# Autodesk Inventor assembly: mg996 3mm top
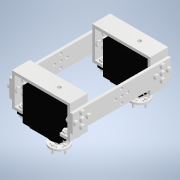
[picture p0: Inventor's stored thumbnail of the model, 180x180]
Saved by Autodesk Inventor 2021.4 (Build 254397000, 397)
## iProperties
Created: 2022-07-09
Part Number: mg996 3mm top
Document SubType Name: Assembly
Designer: isamu
Author: isamu
## Documents named in this file (5)
- D:\personal_projects\robot\inventor\2021\mg996 3mm top.iam
- D:\personal_projects\robot\inventor\2021\base mg996r 3mm frame.iam
- D:\personal_projects\robot\exports\frames\servo frame part 4.ipt
- D:\personal_projects\robot\exports\screws\m3x8.ipt
- D:\personal_projects\robot\exports\screws\m3 nuts.ipt
## Components (44 placed, 4 different names)
1. base mg996r 3mm frame:1 [sub-assembly] — Mate:4, Mate:5, Mate:6, Mate:7, Mate:8, Insert:26, Insert:27, Insert:28, Insert:29, Insert:30, Insert:36, Insert:37, Insert:38, Insert:39, Insert:40
2. base mg996r 3mm frame:2 [sub-assembly] — Mate:1, Mate:2, Mate:3, Mate:9, Mate:10, Mate:11, Insert:21, Insert:22, Insert:23, Insert:24, Insert:25, Insert:31, Insert:32, Insert:33, Insert:34, Insert:35
3. servo frame part 4:1 — Mate:1, Mate:2, Mate:3, Mate:4, Mate:5, Mate:6, Insert:1, Insert:2, Insert:3, Insert:4, Insert:5, Insert:6, Insert:7, Insert:8, Insert:9, Insert:10
4. servo frame part 4:2 — Mate:7, Mate:8, Mate:9, Mate:10, Mate:11, Insert:11, Insert:12, Insert:13, Insert:14, Insert:15, Insert:16, Insert:17, Insert:18, Insert:19, Insert:20
5. m3x8:1 — Insert:5
6. m3x8:2 — Insert:3
7. m3x8:3 — Insert:4
8. m3x8:4 — Insert:1
9. m3x8:5 — Insert:2
10. m3x8:6 — Insert:6
11. m3x8:7 — Insert:7
12. m3x8:8 — Insert:8
13. m3x8:9 — Insert:9
14. m3x8:10 — Insert:10
15. m3x8:11 — Insert:11
16. m3x8:12 — Insert:12
17. m3x8:13 — Insert:13
18. m3x8:14 — Insert:14
19. m3x8:15 — Insert:15
20. m3x8:16 — Insert:17
21. m3x8:17 — Insert:18
22. m3x8:18 — Insert:19
23. m3x8:19 — Insert:20
24. m3x8:20 — Insert:16
25. m3 nuts:1 — Insert:24
26. m3 nuts:2 — Insert:25
27. m3 nuts:3 — Insert:32
28. m3 nuts:4 — Insert:31
29. m3 nuts:5 — Insert:21
30. m3 nuts:6 — Insert:33
31. m3 nuts:7 — Insert:34
32. m3 nuts:8 — Insert:35
33. m3 nuts:9 — Insert:23
34. m3 nuts:10 — Insert:22
35. m3 nuts:11 — Insert:28
36. m3 nuts:12 — Insert:27
37. m3 nuts:13 — Insert:30
38. m3 nuts:14 — Insert:29
39. m3 nuts:15 — Insert:26
40. m3 nuts:16 — Insert:36
41. m3 nuts:17 — Insert:38
42. m3 nuts:18 — Insert:39
43. m3 nuts:19 — Insert:40
44. m3 nuts:20 — Insert:37
## Relationships (51: Insert 40, Mate 11)
- Mate:1: base mg996r 3mm frame:2 ↔ servo frame part 4:1
- Mate:2: base mg996r 3mm frame:2 ↔ servo frame part 4:1
- Mate:3: base mg996r 3mm frame:2 ↔ servo frame part 4:1
- Mate:4: base mg996r 3mm frame:1 ↔ servo frame part 4:1
- Mate:5: base mg996r 3mm frame:1 ↔ servo frame part 4:1
- Mate:6: base mg996r 3mm frame:1 ↔ servo frame part 4:1
- Mate:7: base mg996r 3mm frame:1 ↔ servo frame part 4:2
- Mate:8: base mg996r 3mm frame:1 ↔ servo frame part 4:2
- Mate:9: base mg996r 3mm frame:2 ↔ servo frame part 4:2
- Mate:10: base mg996r 3mm frame:2 ↔ servo frame part 4:2
- Mate:11: base mg996r 3mm frame:2 ↔ servo frame part 4:2
- Insert:1: servo frame part 4:1 ↔ m3x8:4
- Insert:2: servo frame part 4:1 ↔ m3x8:5
- Insert:3: servo frame part 4:1 ↔ m3x8:2
- Insert:4: servo frame part 4:1 ↔ m3x8:3
- Insert:5: servo frame part 4:1 ↔ m3x8:1
- Insert:6: servo frame part 4:1 ↔ m3x8:6
- Insert:7: servo frame part 4:1 ↔ m3x8:7
- Insert:8: servo frame part 4:1 ↔ m3x8:8
- Insert:9: servo frame part 4:1 ↔ m3x8:9
- Insert:10: servo frame part 4:1 ↔ m3x8:10
- Insert:11: servo frame part 4:2 ↔ m3x8:11
- Insert:12: servo frame part 4:2 ↔ m3x8:12
- Insert:13: servo frame part 4:2 ↔ m3x8:13
- Insert:14: servo frame part 4:2 ↔ m3x8:14
- Insert:15: servo frame part 4:2 ↔ m3x8:15
- Insert:16: servo frame part 4:2 ↔ m3x8:20
- Insert:17: servo frame part 4:2 ↔ m3x8:16
- Insert:18: servo frame part 4:2 ↔ m3x8:17
- Insert:19: servo frame part 4:2 ↔ m3x8:18
- Insert:20: servo frame part 4:2 ↔ m3x8:19
- Insert:21: base mg996r 3mm frame:2 ↔ m3 nuts:5
- Insert:22: base mg996r 3mm frame:2 ↔ m3 nuts:10
- Insert:23: base mg996r 3mm frame:2 ↔ m3 nuts:9
- Insert:24: base mg996r 3mm frame:2 ↔ m3 nuts:1
- Insert:25: base mg996r 3mm frame:2 ↔ m3 nuts:2
- Insert:26: base mg996r 3mm frame:1 ↔ m3 nuts:15
- Insert:27: base mg996r 3mm frame:1 ↔ m3 nuts:12
- Insert:28: base mg996r 3mm frame:1 ↔ m3 nuts:11
- Insert:29: base mg996r 3mm frame:1 ↔ m3 nuts:14
- Insert:30: base mg996r 3mm frame:1 ↔ m3 nuts:13
- Insert:31: base mg996r 3mm frame:2 ↔ m3 nuts:4
- Insert:32: base mg996r 3mm frame:2 ↔ m3 nuts:3
- Insert:33: base mg996r 3mm frame:2 ↔ m3 nuts:6
- Insert:34: base mg996r 3mm frame:2 ↔ m3 nuts:7
- Insert:35: base mg996r 3mm frame:2 ↔ m3 nuts:8
- Insert:36: base mg996r 3mm frame:1 ↔ m3 nuts:16
- Insert:37: base mg996r 3mm frame:1 ↔ m3 nuts:20
- Insert:38: base mg996r 3mm frame:1 ↔ m3 nuts:17
- Insert:39: base mg996r 3mm frame:1 ↔ m3 nuts:18
- Insert:40: base mg996r 3mm frame:1 ↔ m3 nuts:19
